# Autodesk Inventor assembly: 3D_V1.2LineFollower
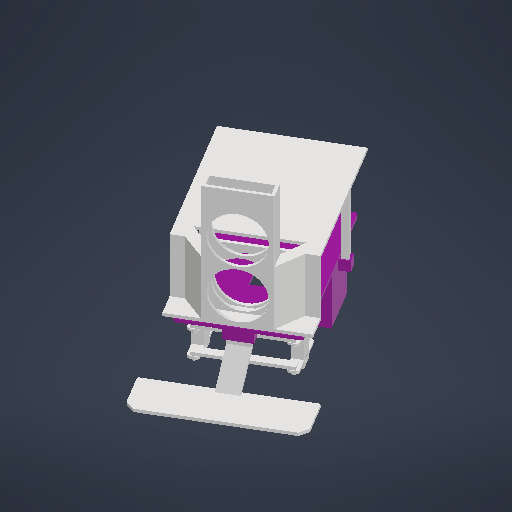
[picture p0: Inventor's stored thumbnail of the model, 512x512]
Saved by Autodesk Inventor 2026.2 (Build 302298000, 298)
## iProperties
Created: 2025-12-14
Part Number: 3D_V1.2LineFollower
Document SubType Name: Assembly
Designer: risda
Author: risda
## Documents named in this file (7)
- C:\Users\risda\OneDrive\Documents\Tugas Kuliah\3D Model Robotika\DesainV1.1\3D_V1.2LineFollower.iam
- C:\Users\risda\OneDrive\Documents\Tugas Kuliah\3D Model Robotika\DesainV1.1\DesainV1.3.ipt
- C:\Users\risda\OneDrive\Documents\Tugas Kuliah\3D Model Robotika\DesainV1.1\DudukanRodaDepan.ipt
- C:\Users\risda\OneDrive\Documents\Tugas Kuliah\3D Model Robotika\DesainV1.1\SteeringWheel.ipt
- C:\Users\risda\OneDrive\Documents\Tugas Kuliah\3D Model Robotika\DesainV1.1\SteeringBaru.ipt
- C:\Users\risda\OneDrive\Documents\Tugas Kuliah\3D Model Robotika\DesainV1.1\DudukanAtas.ipt
- C:\Users\risda\OneDrive\Documents\Tugas Kuliah\3D Model Robotika\DesainV1.1\DudukanLineSensor.ipt
## Components (9 placed, 6 different names)
1. DesainV1.3:1 — Mate:1, Mate:2, Flush:1, Flush:2, Mate:14, Mate:15, Mate:16, Mate:18, Mate:19, Mate:20
2. DudukanRodaDepan:1 — Mate:1, Mate:4, Mate:5, Mate:7, Flush:1, Mate:9, Mate:10, Mate:13, Mate:17
3. DudukanRodaDepan:2 — Mate:2, Mate:3, Mate:6, Flush:2, Mate:8, Mate:11, Mate:12
4. SteeringWheel:1 — Mate:3, Mate:4, Mate:7
5. SteeringWheel:2 — Mate:9, Mate:10, Mate:11
6. SteeringWheel:4 — Mate:5, Mate:6, Mate:8
7. SteeringBaru:1 — Mate:12, Mate:13, Mate:17
8. DudukanAtas:1 — Mate:14, Mate:15, Mate:16
9. DudukanLineSensor:1 — Mate:18, Mate:19, Mate:20
## Relationships (22: Mate 20, Flush 2)
- Mate:1: DesainV1.3:1 ↔ DudukanRodaDepan:1
- Mate:2: DesainV1.3:1 ↔ DudukanRodaDepan:2
- Mate:3: DudukanRodaDepan:2 ↔ SteeringWheel:1
- Mate:4: DudukanRodaDepan:1 ↔ SteeringWheel:1
- Mate:5: DudukanRodaDepan:1 ↔ SteeringWheel:4
- Mate:6: DudukanRodaDepan:2 ↔ SteeringWheel:4
- Mate:7: DudukanRodaDepan:1 ↔ SteeringWheel:1
- Flush:1: DesainV1.3:1 ↔ DudukanRodaDepan:1
- Flush:2: DesainV1.3:1 ↔ DudukanRodaDepan:2
- Mate:8: DudukanRodaDepan:2 ↔ SteeringWheel:4
- Mate:9: DudukanRodaDepan:1 ↔ SteeringWheel:2
- Mate:10: DudukanRodaDepan:1 ↔ SteeringWheel:2
- Mate:11: DudukanRodaDepan:2 ↔ SteeringWheel:2
- Mate:12: DudukanRodaDepan:2 ↔ SteeringBaru:1
- Mate:13: DudukanRodaDepan:1 ↔ SteeringBaru:1
- Mate:14: DesainV1.3:1 ↔ DudukanAtas:1
- Mate:15: DesainV1.3:1 ↔ DudukanAtas:1
- Mate:16: DesainV1.3:1 ↔ DudukanAtas:1
- Mate:17: DudukanRodaDepan:1 ↔ SteeringBaru:1
- Mate:18: DesainV1.3:1 ↔ DudukanLineSensor:1
- Mate:19: DesainV1.3:1 ↔ DudukanLineSensor:1
- Mate:20: DesainV1.3:1 ↔ DudukanLineSensor:1
